# Autodesk Inventor assembly: COTS_GENERIC_LED_Strip_399mm
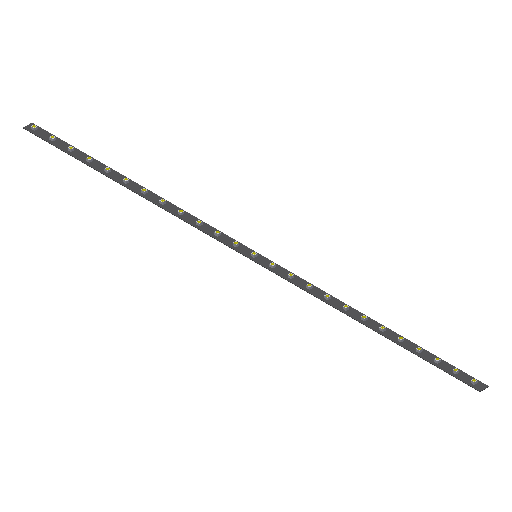
[picture p0: Inventor's stored thumbnail of the model, 512x512]
Saved by Autodesk Inventor 2026.1 (Build 301233000, 233)
## iProperties
Created: 2016-06-18
Part Number: COTS_GENERIC_LED_Strip_399mm
Material: Ogólny
Document SubType Name: Assembly
Designer: Andrzej
Mass: 1.3671 g
Surface Area: 76.2259 cm^2
Volume: 1.3671 cm^3
Density: 1 g/cm^3
Author: Andrzej
## Documents named in this file (4)
- C:\Users\Andrzej\OneDrive\_DRIVE_SYNCH_FILES\__ BYTECHLAB PROJECTS\MECH - FDM 3D Printer - RAPTOR-360\MCAD\1_REV1\__COTS_PARTS\COTS_GENERIC_LED_Strip_399mm\COTS_GENERIC_LED_Strip_399mm.iam
- C:\Users\Andrzej\OneDrive\_DRIVE_SYNCH_FILES\__ BYTECHLAB PROJECTS\MECH - FDM 3D Printer - RAPTOR-360\MCAD\1_REV1\__COTS_PARTS\COTS_GENERIC_LED_Strip_399mm\pasek ledów os x 410mm.ipt
- C:\Users\Andrzej\OneDrive\_DRIVE_SYNCH_FILES\__ BYTECHLAB PROJECTS\MECH - FDM 3D Printer - RAPTOR-360\MCAD\1_REV1\__COTS_PARTS\COTS_GENERIC_LED_Strip_399mm\pasek led 410mm os x zlozony.ipt
- C:\Users\Andrzej\OneDrive\_DRIVE_SYNCH_FILES\__ BYTECHLAB PROJECTS\MECH - FDM 3D Printer - RAPTOR-360\MCAD\1_REV1\__COTS_PARTS\COTS_GENERIC_LED_Strip_399mm\led od paska ledów.ipt
## Components (27 placed, 3 different names)
1. pasek ledów os x 410mm:1 — Równoległy:1, Równoległy:2, Zestawiający:1, Równoległy:3, Równoległy:4
2. pasek led 410mm os x zlozony:1 — Równoległy:1, Równoległy:2
3. led od paska ledów:1 — Zestawiający:1, Równoległy:3, Równoległy:4
4. led od paska ledów:2
5. led od paska ledów:3
6. led od paska ledów:4
7. led od paska ledów:5
8. led od paska ledów:6
9. led od paska ledów:7
10. led od paska ledów:8
11. led od paska ledów:9
12. led od paska ledów:10
13. led od paska ledów:11
14. led od paska ledów:12
15. led od paska ledów:13
16. led od paska ledów:14
17. led od paska ledów:15
18. led od paska ledów:16
19. led od paska ledów:17
20. led od paska ledów:18
21. led od paska ledów:19
22. led od paska ledów:20
23. led od paska ledów:21
24. led od paska ledów:22
25. led od paska ledów:23
26. led od paska ledów:24
27. led od paska ledów:25
## Component patterns: (25 elements, first: led od paska ledów:1)
## Relationships (5: Flush 4, Mate 1)
- Równoległy:1 [Flush]: pasek ledów os x 410mm:1 ↔ pasek led 410mm os x zlozony:1
- Równoległy:2 [Flush]: pasek ledów os x 410mm:1 ↔ pasek led 410mm os x zlozony:1
- Zestawiający:1 [Mate]: pasek ledów os x 410mm:1 ↔ led od paska ledów:1
- Równoległy:3 [Flush] (7.5 mm): pasek ledów os x 410mm:1 ↔ led od paska ledów:1
- Równoległy:4 [Flush] (2.625 mm): pasek ledów os x 410mm:1 ↔ led od paska ledów:1
